# Autodesk Inventor assembly: Linear_stretcher
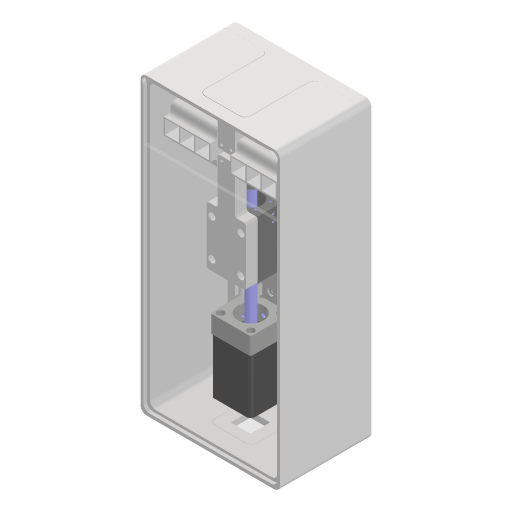
[picture p0: Inventor's stored thumbnail of the model, 512x512]
Saved by Autodesk Inventor 2023 (Build 270158000, 158)
## iProperties
Company: ZWCAD Software Co.
Created: 2026-04-09
Part Number: Linear_stretcher
Description: This file contains a STEP AP42 implementation
Document SubType Name: Assembly
Designer: ferrerx
Sending System: ZW3D to STEP translator
Preprocessor: Version 1.0
Title: PDM35E247-BS0802-1.5-4-40-001.stp
Revision Number: ANYUNSPECIFIED
## Documents named in this file (23)
- C:\Users\ferrerx\The Francis Crick Dropbox\MakingLab\Projects\MSTP00412 - Linear cell stretcher\Linear_stretcher.iam
- C:\Users\ferrerx\The Francis Crick Dropbox\MakingLab\Projects\MSTP00412 - Linear cell stretcher\16-35-901.ipt
- C:\Users\ferrerx\The Francis Crick Dropbox\MakingLab\Projects\MSTP00412 - Linear cell stretcher\28-35-001.iam
- C:\Users\ferrerx\The Francis Crick Dropbox\MakingLab\Projects\MSTP00412 - Linear cell stretcher\16-35-902.ipt
- C:\Users\ferrerx\The Francis Crick Dropbox\MakingLab\Projects\MSTP00412 - Linear cell stretcher\16-42-914.ipt
- C:\Users\ferrerx\The Francis Crick Dropbox\MakingLab\Projects\MSTP00412 - Linear cell stretcher\12-015.ipt
- C:\Users\ferrerx\The Francis Crick Dropbox\MakingLab\Projects\MSTP00412 - Linear cell stretcher\03-42-914.ipt
- C:\Users\ferrerx\The Francis Crick Dropbox\MakingLab\Projects\MSTP00412 - Linear cell stretcher\03-42-916.ipt
- C:\Users\ferrerx\The Francis Crick Dropbox\MakingLab\Projects\MSTP00412 - Linear cell stretcher\09-28-002.ipt
- C:\Users\ferrerx\The Francis Crick Dropbox\MakingLab\Projects\MSTP00412 - Linear cell stretcher\11-003.ipt
- C:\Users\ferrerx\The Francis Crick Dropbox\MakingLab\Projects\MSTP00412 - Linear cell stretcher\16-35-903.ipt
- C:\Users\ferrerx\The Francis Crick Dropbox\MakingLab\Projects\MSTP00412 - Linear cell stretcher\B35E247-0-1.5-4-STD.ipt
- C:\Users\ferrerx\The Francis Crick Dropbox\MakingLab\Projects\MSTP00412 - Linear cell stretcher\16-35-904.ipt
- C:\Users\ferrerx\The Francis Crick Dropbox\MakingLab\Projects\MSTP00412 - Linear cell stretcher\12-004.ipt
- C:\Users\ferrerx\The Francis Crick Dropbox\MakingLab\Projects\MSTP00412 - Linear cell stretcher\21-42-903.ipt
- C:\Users\ferrerx\The Francis Crick Dropbox\MakingLab\Projects\MSTP00412 - Linear cell stretcher\Beam breaker.ipt
- C:\Users\ferrerx\The Francis Crick Dropbox\MakingLab\Projects\MSTP00412 - Linear cell stretcher\Enclosure base.ipt
- C:\Users\ferrerx\The Francis Crick Dropbox\MakingLab\Projects\MSTP00412 - Linear cell stretcher\Puller.ipt
- C:\Users\ferrerx\The Francis Crick Dropbox\MakingLab\Projects\MSTP00412 - Linear cell stretcher\Rod.ipt
- C:\Users\ferrerx\The Francis Crick Dropbox\MakingLab\Projects\MSTP00412 - Linear cell stretcher\Well.ipt
- C:\Users\ferrerx\The Francis Crick Dropbox\MakingLab\Projects\MSTP00412 - Linear cell stretcher\Eclosure lid.ipt
- C:\Users\ferrerx\The Francis Crick Dropbox\MakingLab\Projects\MSTP00412 - Linear cell stretcher\PMMA_lid.ipt
- C:\Users\ferrerx\The Francis Crick Dropbox\MakingLab\Projects\MSTP00412 - Linear cell stretcher\PMMA_lid_long.ipt
## Components (25 placed, 22 different names)
1. 16-35-901 — Mate:13, Mate:14, Mate:19, Mate:26
2. 28-35-001 [sub-assembly] — Mate:18, Mate:39, Mate:40, Mate:53
3. 16-35-902 — Mate:1, Mate:2, Mate:3, Mate:4, Flush:1, Mate:20, Mate:21, Mate:22
4. 16-42-914 — Mate:39, Mate:40, Mate:41, Mate:42, Mate:43, Mate:44, Mate:45, Mate:46, Mate:47, Mate:48, Mate:49
5. 03-42-914 — Mate:5, Mate:6, Mate:7, Mate:12, Mate:43
6. 03-42-916 — Mate:41, Mate:42
7. 09-28-002 — Mate:2, Mate:6, Flush:1, Mate:8
8. 11-003 — Mate:5, Mate:7, Mate:8
9. 16-35-903 — Mate:1, Mate:3, Mate:4, Mate:18, Mate:19, Mate:30, Mate:31, Mate:32, Mate:53
10. B35E247-0-1 — Mate:12, Mate:13, Mate:14, Mate:26
11. 16-35-904 — Mate:25
12. 12-004 — Mate:25
13. 12-004:1
14. 21-42-903 — Mate:20, Mate:21, Mate:22
15. 12-015:4
16. Beam breaker:1 — Mate:44, Mate:45, Mate:46
17. Enclosure base:1 — Mate:30, Mate:31, Mate:32, Mate:54, Mate:55
18. Puller:1 — Mate:47, Mate:48, Mate:49, Mate:50, Flush:2
19. Rod:1 — Mate:37, Mate:38, Mate:50, Flush:2, Flush:3
20. Well:1 — Mate:37, Mate:51
21. Well:2 — Mate:38, Mate:52
22. Rod:2 — Mate:51, Mate:52, Flush:3
23. Eclosure lid:1 — Mate:54, Mate:55, Mate:56, Mate:57, Mate:58, Mate:59, Mate:60, Mate:61
24. PMMA_lid:1 — Mate:59, Mate:60, Mate:61
25. PMMA_lid_long:1 — Mate:56, Mate:57, Mate:58
## Relationships (49: Mate 46, Flush 3)
- Mate:1: 16-35-902 ↔ 16-35-903
- Mate:2: 16-35-902 ↔ 09-28-002
- Mate:3: 16-35-902 ↔ 16-35-903
- Mate:4: 16-35-902 ↔ 16-35-903
- Mate:5: 03-42-914 ↔ 11-003
- Mate:6: 03-42-914 ↔ 09-28-002
- Mate:7: 03-42-914 ↔ 11-003
- Flush:1: 16-35-902 ↔ 09-28-002
- Mate:8: 09-28-002 ↔ 11-003
- Mate:12: 03-42-914 ↔ B35E247-0-1
- Mate:13: 16-35-901 ↔ B35E247-0-1
- Mate:14: 16-35-901 ↔ B35E247-0-1
- Mate:18: 28-35-001 ↔ 16-35-903
- Mate:19: 16-35-901 ↔ 16-35-903
- Mate:20: 16-35-902 ↔ 21-42-903
- Mate:21: 16-35-902 ↔ 21-42-903
- Mate:22: 16-35-902 ↔ 21-42-903
- Mate:25: 16-35-904 ↔ 12-004
- Mate:26: 16-35-901 ↔ B35E247-0-1
- Mate:30: 16-35-903 ↔ Enclosure base:1
- Mate:31: 16-35-903 ↔ Enclosure base:1
- Mate:32: 16-35-903 ↔ Enclosure base:1
- Mate:37: Rod:1 ↔ Well:1
- Mate:38: Rod:1 ↔ Well:2
- Mate:39: 28-35-001 ↔ 16-42-914
- Mate:40: 28-35-001 ↔ 16-42-914
- Mate:41: 16-42-914 ↔ 03-42-916
- Mate:42: 16-42-914 ↔ 03-42-916
- Mate:43: 16-42-914 ↔ 03-42-914
- Mate:44: 16-42-914 ↔ Beam breaker:1
- Mate:45: 16-42-914 ↔ Beam breaker:1
- Mate:46: 16-42-914 ↔ Beam breaker:1
- Mate:47: 16-42-914 ↔ Puller:1
- Mate:48: 16-42-914 ↔ Puller:1
- Mate:49: 16-42-914 ↔ Puller:1
- Mate:50: Puller:1 ↔ Rod:1
- Flush:2 (-42.5 mm): Puller:1 ↔ Rod:1
- Mate:51: Well:1 ↔ Rod:2
- Mate:52: Well:2 ↔ Rod:2
- Flush:3: Rod:1 ↔ Rod:2
- Mate:53: 28-35-001 ↔ 16-35-903
- Mate:54: Enclosure base:1 ↔ Eclosure lid:1
- Mate:55: Enclosure base:1 ↔ Eclosure lid:1
- Mate:56: Eclosure lid:1 ↔ PMMA_lid_long:1
- Mate:57: Eclosure lid:1 ↔ PMMA_lid_long:1
- Mate:58: Eclosure lid:1 ↔ PMMA_lid_long:1
- Mate:59: Eclosure lid:1 ↔ PMMA_lid:1
- Mate:60: Eclosure lid:1 ↔ PMMA_lid:1
- Mate:61: Eclosure lid:1 ↔ PMMA_lid:1
